# Autodesk Inventor assembly: LidarTilt
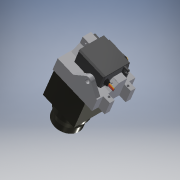
[picture p0: Inventor's stored thumbnail of the model, 180x180]
Saved by Autodesk Inventor 2017 (Build 210142000, 142)
## iProperties
Created: 2017-03-20
Part Number: LidarTilt
Document SubType Name: Assembly
Designer: Naga
Author: Naga
## Documents named in this file (4)
- E:\GDrive\IEEE CS\SoutheastCon2017\Cad\Electronics\LidarTilt.iam
- E:\GDrive\IEEE CS\SoutheastCon2017\Cad\Electronics\Lidar.ipt
- E:\GDrive\IEEE CS\SoutheastCon2017\Cad\tilt\tiltLidarMount.ipt
- E:\GDrive\IEEE CS\SoutheastCon2017\Cad\Motors\MG995_Servo.iam
## Components (3 placed, 3 different names)
1. Lidar:1 — Flush:1, Flush:2, Mate:5
2. tiltLidarMount:1 — Flush:1, Flush:2, Mate:3, Mate:4, Mate:5, Mate:6
3. MG995_Servo:1 [sub-assembly] — Mate:3, Mate:4, Mate:6
## Relationships (6: Mate 4, Flush 2)
- Flush:1: Lidar:1 ↔ tiltLidarMount:1
- Flush:2 (3.2893 mm): Lidar:1 ↔ tiltLidarMount:1
- Mate:3: tiltLidarMount:1 ↔ MG995_Servo:1
- Mate:4: tiltLidarMount:1 ↔ MG995_Servo:1
- Mate:5: Lidar:1 ↔ tiltLidarMount:1
- Mate:6: tiltLidarMount:1 ↔ MG995_Servo:1
